# Autodesk Inventor assembly: BuiltV1
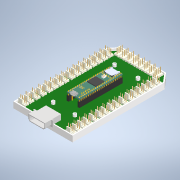
[picture p0: Inventor's stored thumbnail of the model, 180x180]
Saved by Autodesk Inventor 2021 (Build 250183000, 183)
## iProperties
Created: 2021-02-27
Part Number: BuiltV1
Document SubType Name: Assembly
Designer: Collin
Author: Collin
## Documents named in this file (5)
- H:\Projects\RGB Controller\Teensy-PC_RGB_Controller\2 PCB\CAD\BuiltV1.iam
- H:\Projects\RGB Controller\Teensy-PC_RGB_Controller\2 PCB\CAD\CaseV1.ipt
- H:\Projects\RGB Controller\Teensy-PC_RGB_Controller\2 PCB\CAD\CircuitBoard.iam
- H:\Projects\RGB Controller\Teensy-PC_RGB_Controller\2 PCB\CAD\teensy-4-1-development-board-1.snapshot.5\Teensy 4.1 (With Headers).iam
- H:\Projects\RGB Controller\Teensy-PC_RGB_Controller\2 PCB\CAD\MolexConnector.ipt
## Components (4 placed, 4 different names)
1. CaseV1:1 — Mate:1, Mate:2, Mate:3, Mate:7, Angle:1, Mate:9
2. CircuitBoard:1 [sub-assembly] — Mate:1, Mate:2, Mate:3, Mate:4, Mate:5, Mate:6, Mate:7
3. Teensy 4.1 (With Headers):1 [sub-assembly] — Mate:4, Mate:5, Mate:6, Flush:1
4. MolexConnector:1 — Angle:1, Mate:9, Flush:1
## Relationships (10: Mate 8, Angle 1, Flush 1)
- Mate:1: CaseV1:1 ↔ CircuitBoard:1
- Mate:2: CaseV1:1 ↔ CircuitBoard:1
- Mate:3: CaseV1:1 ↔ CircuitBoard:1
- Mate:4: CircuitBoard:1 ↔ Teensy 4.1 (With Headers):1
- Mate:5: CircuitBoard:1 ↔ Teensy 4.1 (With Headers):1
- Mate:6: CircuitBoard:1 ↔ Teensy 4.1 (With Headers):1
- Mate:7: CaseV1:1 ↔ CircuitBoard:1
- Angle:1 (0 deg): CaseV1:1 ↔ MolexConnector:1
- Mate:9: CaseV1:1 ↔ MolexConnector:1
- Flush:1: Teensy 4.1 (With Headers):1 ↔ MolexConnector:1
